# Autodesk Inventor assembly: quad_bai_t_sim
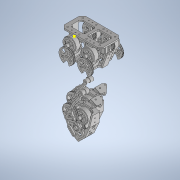
[picture p0: Inventor's stored thumbnail of the model, 180x180]
Saved by Autodesk Inventor 2020 (Build 240168000, 168)
## iProperties
Created: 2021-03-10
Part Number: quad_bai_t_sim
Document SubType Name: Assembly
Designer: Shuang Peng
Author: Shuang Peng
## Documents named in this file (5)
- D:\projects-3\biped_tiny\hardware\sim_mod\quad_bai_t_sim.iam
- D:\projects-3\biped_tiny\hardware\body_shell_1.ipt
- D:\projects-3\biped_tiny\hardware\body_shell_2.ipt
- D:\projects-3\biped_tiny\hardware\sim_mod\reducer_1.iam
- D:\projects-3\biped_tiny\hardware\sim_mod\leg_1_sim.iam
## Components (8 placed, 4 different names)
1. body_shell_1:1 — Insert:1, Insert:2, Insert:3, Insert:4, Insert:5, Insert:6, Insert:7, Insert:8, Insert:9, Insert:10
2. body_shell_2:1 — Mate:1, Mate:2, Insert:1, Insert:2
3. reducer_1:1 [sub-assembly] — Insert:9, Insert:10
4. reducer_1:2 [sub-assembly] — Insert:7, Insert:8
5. reducer_1:3 [sub-assembly] — Insert:5, Insert:6
6. reducer_1:4 [sub-assembly] — Insert:3, Insert:4
7. leg_1_sim:1 [sub-assembly]
8. leg_1_sim:2 [sub-assembly]
## Relationships (12: Insert 10, Mate 2)
- Mate:1: body_shell_2:1
- Mate:2: body_shell_2:1
- Insert:1: body_shell_1:1 ↔ body_shell_2:1
- Insert:2: body_shell_1:1 ↔ body_shell_2:1
- Insert:3: body_shell_1:1 ↔ reducer_1:4
- Insert:4: body_shell_1:1 ↔ reducer_1:4
- Insert:5: body_shell_1:1 ↔ reducer_1:3
- Insert:6: body_shell_1:1 ↔ reducer_1:3
- Insert:7: body_shell_1:1 ↔ reducer_1:2
- Insert:8: body_shell_1:1 ↔ reducer_1:2
- Insert:9: body_shell_1:1 ↔ reducer_1:1
- Insert:10: body_shell_1:1 ↔ reducer_1:1
